# Autodesk Inventor assembly: AM-2235
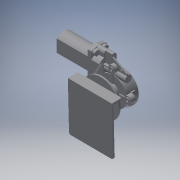
[picture p0: Inventor's stored thumbnail of the model, 180x180]
Saved by Autodesk Inventor 2016 (Build 200138000, 138)
## iProperties
Created: 2012-12-12
Part Number: AM-2235
Description: STEP AP203
Document SubType Name: Assembly
Designer: bbier
Sending System: SolidWorks 2010
Preprocessor: SwSTEP 2.0
Title: AM-2235.STEP
Revision Number: ANY
## Documents named in this file (9)
- C:\Users\bbier\OneDrive\Documents\Snobotics\Robot2016\chassis\version2\AM-2235.iam
- C:\Users\bbier\OneDrive\Documents\Snobotics\CAD\Standard Parts\Motors\AM-2235 output shaft.ipt
- C:\Users\bbier\OneDrive\Documents\Snobotics\CAD\Standard Parts\Motors\AM-2235 gearbox housing.ipt
- C:\Users\bbier\OneDrive\Documents\Snobotics\CAD\Standard Parts\Motors\AM-2235 threaded insert.ipt
- C:\Users\bbier\OneDrive\Documents\Snobotics\CAD\Standard Parts\Motors\AM-2235 motor.ipt
- C:\Users\bbier\OneDrive\Documents\Snobotics\CAD\Standard Parts\Motors\AM-2235 gear cap.ipt
- C:\Users\bbier\OneDrive\Documents\Snobotics\CAD\Standard Parts\Motors\am-2279+10mm+DD+Bore+Hub.ipt
- C:\Users\bbier\OneDrive\Documents\Snobotics\Robot2016\chassis\version2\sprocket.ipt
- C:\Users\bbier\OneDrive\Documents\Snobotics\Robot2016\chassis\version2\snoBlowerBracket.ipt
## Components (10 placed, 10 different names)
1. AM-2235 output shaft_1 — Mate:2, Flush:1
2. AM-2235 gearbox housing_2
3. AM-2235 threaded insert_3
4. AM-2235 motor_4
5. AM-2235 threaded insert_5
6. AM-2235 threaded insert_6
7. AM-2235 gear cap_7
8. am-2279+10mm+DD+Bore+Hub:1 — Mate:2, Flush:1, Mate:3, Mate:4
9. sprocket:1 — Mate:3, Mate:4
10. snoBlowerBracket:1
## Relationships (4: Mate 3, Flush 1)
- Mate:2: AM-2235 output shaft_1 ↔ am-2279+10mm+DD+Bore+Hub:1
- Flush:1: AM-2235 output shaft_1 ↔ am-2279+10mm+DD+Bore+Hub:1
- Mate:3: am-2279+10mm+DD+Bore+Hub:1 ↔ sprocket:1
- Mate:4: am-2279+10mm+DD+Bore+Hub:1 ↔ sprocket:1
